# Autodesk Inventor assembly: Zusammenbau
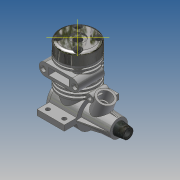
[picture p0: Inventor's stored thumbnail of the model, 180x180]
Saved by Autodesk Inventor 2021 (Build 250183000, 183)
## iProperties
Created: 2021-01-14
Part Number: Zusammenbau
Document SubType Name: Assembly
Designer: Sander
Author: Sander
## Documents named in this file (13)
- C:\Users\ricar\OneDrive - Fachhochschule Aachen\Mechatronik I\CAD\INVENTOR\Proyectos\Daten\Zusammenbau.iam
- C:\Users\ricar\OneDrive - Fachhochschule Aachen\Mechatronik I\CAD\INVENTOR\Proyectos\Daten\Motorblock_ra8846s.ipt
- C:\Users\ricar\OneDrive - Fachhochschule Aachen\Mechatronik I\CAD\INVENTOR\Proyectos\Daten\Zylinderkopf_ra8846s.ipt
- C:\Users\ricar\OneDrive - Fachhochschule Aachen\Mechatronik I\CAD\INVENTOR\Proyectos\Daten\Gehäusedeckel_ra8846s.ipt
- C:\Users\ricar\OneDrive - Fachhochschule Aachen\Mechatronik I\CAD\INVENTOR\Proyectos\Daten\Zylinderbuchse_ra8846s.ipt
- C:\Users\ricar\OneDrive - Fachhochschule Aachen\Mechatronik I\CAD\INVENTOR\Proyectos\Daten\Zylinderbuchsenring_ra8846s.ipt
- C:\Users\ricar\OneDrive - Fachhochschule Aachen\Mechatronik I\CAD\INVENTOR\Proyectos\Daten\Schlitzschraube_ra8846s\Schlitzschraube_ra8846s-01.ipt
- C:\Users\ricar\OneDrive - Fachhochschule Aachen\Mechatronik I\CAD\INVENTOR\Proyectos\Daten\Schlitzschraube_ra8846s.ipt
- C:\Users\ricar\OneDrive - Fachhochschule Aachen\Mechatronik I\CAD\INVENTOR\Proyectos\Daten\Unterlegescheibe_ra8846s.ipt
- C:\Users\ricar\OneDrive - Fachhochschule Aachen\Mechatronik I\CAD\INVENTOR\Proyectos\Daten\Kurbelwelle_ra8846s.ipt
- C:\Users\ricar\OneDrive - Fachhochschule Aachen\Mechatronik I\CAD\INVENTOR\Proyectos\Daten\Kolben_ra8846s.ipt
- C:\Users\ricar\OneDrive - Fachhochschule Aachen\Mechatronik I\CAD\INVENTOR\Proyectos\Daten\Kolbenbolzen_ra8846s.ipt
- C:\Users\ricar\OneDrive - Fachhochschule Aachen\Mechatronik I\CAD\INVENTOR\Proyectos\Daten\Pleuel_ra8846s.ipt
## Components (14 placed, 11 different names)
1. Motorblock_ra8846s:1 — Einfügen:1, Einfügen:2, Einfügen:3, Einfügen:4, Einfügen:6
2. Zylinderkopf_ra8846s:1 — Einfügen:1, Einfügen:5
3. Gehäusedeckel_ra8846s:1 — Einfügen:2
4. Zylinderbuchse_ra8846s:1 — Einfügen:3, Passend:3
5. Zylinderbuchsenring_ra8846s:1 — Einfügen:4
6. Unterlegescheibe_ra8846s:1 — Einfügen:6, Einfügen:7
7. Kurbelwelle_ra8846s:1 — Einfügen:7, Passend:4
8. Kolben_ra8846s:1 — Passend:1, Passend:2, Passend:3
9. Kolbenbolzen_ra8846s:1 — Passend:1, Passend:2, Passend:5
10. Pleuel_ra8846s:1 — Passend:4, Passend:5
11. Schlitzschraube_ra8846s-01:1 — Einfügen:5
12. Schlitzschraube_ra8846s-01:2
13. Schlitzschraube_ra8846s-01:3
14. Schlitzschraube_ra8846s-01:4
## Component patterns: (4 elements, first: Schlitzschraube_ra8846s-01:1)
## Relationships (12: Insert 7, Mate 5)
- Einfügen:1 [Insert]: Motorblock_ra8846s:1 ↔ Zylinderkopf_ra8846s:1
- Einfügen:2 [Insert]: Motorblock_ra8846s:1 ↔ Gehäusedeckel_ra8846s:1
- Einfügen:3 [Insert]: Motorblock_ra8846s:1 ↔ Zylinderbuchse_ra8846s:1
- Einfügen:4 [Insert]: Motorblock_ra8846s:1 ↔ Zylinderbuchsenring_ra8846s:1
- Einfügen:5 [Insert]: Zylinderkopf_ra8846s:1 ↔ Schlitzschraube_ra8846s-01:1
- Einfügen:6 [Insert]: Motorblock_ra8846s:1 ↔ Unterlegescheibe_ra8846s:1
- Einfügen:7 [Insert]: Unterlegescheibe_ra8846s:1 ↔ Kurbelwelle_ra8846s:1
- Passend:1 [Mate]: Kolben_ra8846s:1 ↔ Kolbenbolzen_ra8846s:1
- Passend:2 [Mate] (-6 mm): Kolben_ra8846s:1 ↔ Kolbenbolzen_ra8846s:1
- Passend:3 [Mate]: Zylinderbuchse_ra8846s:1 ↔ Kolben_ra8846s:1
- Passend:4 [Mate]: Kurbelwelle_ra8846s:1 ↔ Pleuel_ra8846s:1
- Passend:5 [Mate]: Kolbenbolzen_ra8846s:1 ↔ Pleuel_ra8846s:1
